# Autodesk Inventor assembly: RotorAssembly
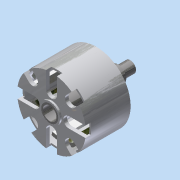
[picture p0: Inventor's stored thumbnail of the model, 180x180]
Saved by Autodesk Inventor 2015 (Build 190159000, 159)
## iProperties
Created: 2015-12-24
Part Number: RotorAssembly
Document SubType Name: Assembly
Designer: Raphael
Author: Raphael
## Documents named in this file (3)
- \\psf\Home\Documents\electric-skateboard\CAD\HubMotor\RotorAssembly.iam
- \\psf\Home\Documents\electric-skateboard\CAD\HubMotor\OuterShaft.ipt
- \\psf\Home\Documents\electric-skateboard\CAD\HubMotor\Rotor.ipt
## Components (2 placed, 2 different names)
1. OuterShaft:1 — Mate:1, Flush:1
2. Rotor:1 — Mate:1, Flush:1
## Relationships (2: Mate 1, Flush 1)
- Mate:1: OuterShaft:1 ↔ Rotor:1
- Flush:1: OuterShaft:1 ↔ Rotor:1
